# Autodesk Inventor assembly: V4
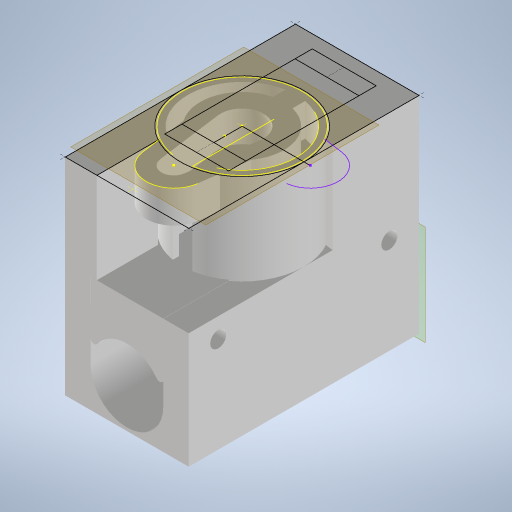
[picture p0: Inventor's stored thumbnail of the model, 512x512]
Saved by Autodesk Inventor 2024 (Build 280153000, 153)
## iProperties
Created: 2024-11-24
Part Number: V4
Document SubType Name: Assembly
Designer: Tommy Rohmann
Author: Tommy Rohmann
## Documents named in this file (4)
- C:\Users\Tommy Rohmann\OneDrive\Projects\Microgravity-Press-Washing-Machine\System Design and Documentation\Piping Systems\Actuated Ball Valves\V4.iam
- C:\Users\Tommy Rohmann\OneDrive\Projects\Microgravity-Press-Washing-Machine\System Design and Documentation\Piping Systems\Actuated Ball Valves\Ball Valve Mount 4.ipt
- C:\Users\Tommy Rohmann\OneDrive\Projects\Microgravity-Press-Washing-Machine\System Design and Documentation\Piping Systems\Actuated Ball Valves\Servo Adapter 4.ipt
- C:\Users\Tommy Rohmann\OneDrive\Projects\Microgravity-Press-Washing-Machine\System Design and Documentation\Piping Systems\Actuated Ball Valves\Servo Mount V4.ipt
## Components (3 placed, 3 different names)
1. Ball Valve Mount 4:1 — Mate:1, Mate:2, Angle:1, Flush:3
2. Servo Adapter 4:1 — Mate:1, Mate:2, Angle:1, Flush:1, Flush:2
3. Servo Mount V4:1 — Flush:1, Flush:2, Flush:3
## Relationships (6: Flush 3, Mate 2, Angle 1)
- Mate:1: Ball Valve Mount 4:1 ↔ Servo Adapter 4:1
- Mate:2: Ball Valve Mount 4:1 ↔ Servo Adapter 4:1
- Angle:1 (0 deg): Ball Valve Mount 4:1 ↔ Servo Adapter 4:1
- Flush:1: Servo Adapter 4:1 ↔ Servo Mount V4:1
- Flush:2: Servo Adapter 4:1 ↔ Servo Mount V4:1
- Flush:3: Ball Valve Mount 4:1 ↔ Servo Mount V4:1
